# Autodesk Inventor assembly: ant-backlash
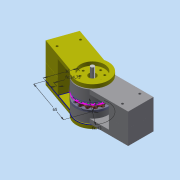
[picture p0: Inventor's stored thumbnail of the model, 180x180]
Saved by Autodesk Inventor 2020.2 (Build 242310000, 310)
## iProperties
Created: 2018-11-17
Part Number: ant-backlash
Document SubType Name: Assembly
Designer: paulg
Author: paulg
## Documents named in this file (13)
- D:\Projects\MiniBot\CAD\cycloidal gear\source\ant-backlash.iam
- D:\Projects\MiniBot\CAD\cycloidal gear\source\ab_output_in.ipt
- D:\Projects\MiniBot\CAD\cycloidal gear\source\ab_output_out.ipt
- D:\Projects\MiniBot\CAD\cycloidal gear\source\Main_equation_fixed_9mm.ipt
- D:\Projects\MiniBot\CAD\cycloidal gear\source\offset 6id 12- od 9mm.ipt
- D:\Projects\MiniBot\CAD\cycloidal gear\source\45x58x7 bearing.ipt
- D:\Projects\MiniBot\CAD\cycloidal gear\source\encoder in 6809_ab.ipt
- D:\Projects\MiniBot\CAD\cycloidal gear\source\motor_6809_ab.ipt
- D:\Projects\MiniBot\CAD\cycloidal gear\source\motor_shaft-ab.ipt
- D:\Projects\MiniBot\CAD\cycloidal gear\source\12x6x4 bearing.ipt
- D:\Projects\MiniBot\CAD\cycloidal gear\source\18x12x4 bearing.ipt
- D:\Projects\MiniBot\CAD\cycloidal gear\source\8x5x2.5 bearing.ipt
- D:\Projects\MiniBot\CAD\cycloidal gear\source\inner_rods.ipt
## Components (40 placed, 12 different names)
1. ab_output_in:1 — Insert:1, Insert:2, Passend:16, Passend:17
2. ab_output_out:1 — Insert:1, Insert:11, Flush:2, Passend:16, Passend:17, Passend:18
3. ab_output_out:2 — Insert:2, Insert:8, Flush:2, Passend:18
4. Main_equation_fixed_9mm:1 — Insert:17, Insert:25, Passend:10, Passend:12
5. offset 6id 12- od 9mm:1 — Insert:5, Insert:22, Insert:24, Passend:6, Passend:7, Passend:8, Passend:9, Passend:10, Passend:11, Passend:12, Passend:13, Passend:14
6. Main_equation_fixed_9mm:2 — Insert:5, Insert:16, Insert:19, Insert:21, Passend:11, Passend:15
7. encoder in 6809_ab:1 — Insert:6, Passend:19
8. motor_6809_ab:1 — Insert:12, Einfügen:23, Passend:5, Passend:19
9. 45x58x7 bearing:1 — Insert:11, Insert:12
10. 45x58x7 bearing:2 — Insert:6, Insert:8
11. motor_shaft-ab:1 — Passend:3, Passend:5, Passend:6
12. 12x6x4 bearing:1 — Passend:3, Passend:7
13. 18x12x4 bearing:1 — Insert:19, Passend:8, Passend:14
14. 18x12x4 bearing:2 — Insert:21, Passend:9, Passend:13, Passend:15
15. 18x12x4 bearing:3 — Insert:22
16. 18x12x4 bearing:4 — Insert:24, Insert:25
17. 8x5x2.5 bearing:2 — Insert:16
18. 8x5x2.5 bearing:3
19. 8x5x2.5 bearing:4
20. 8x5x2.5 bearing:5
21. 8x5x2.5 bearing:6
22. 8x5x2.5 bearing:7
23. 8x5x2.5 bearing:8
24. 8x5x2.5 bearing:9
25. 8x5x2.5 bearing:1 — Insert:17
26. 8x5x2.5 bearing:10
27. 8x5x2.5 bearing:11
28. 8x5x2.5 bearing:12
29. 8x5x2.5 bearing:13
30. 8x5x2.5 bearing:14
31. 8x5x2.5 bearing:15
32. 8x5x2.5 bearing:16
33. inner_rods:1 — Einfügen:23
34. inner_rods:2
35. inner_rods:3
36. inner_rods:4
37. inner_rods:5
38. inner_rods:6
39. inner_rods:7
40. inner_rods:8
## Component patterns: (8 elements, first: 8x5x2.5 bearing:2), (8 elements, first: 8x5x2.5 bearing:1), (8 elements, first: inner_rods:1)
## Relationships (32: Mate 16, Insert 15, Flush 1)
- Insert:1: ab_output_in:1 ↔ ab_output_out:1
- Insert:2: ab_output_in:1 ↔ ab_output_out:2
- Insert:5 (0.5 mm): offset 6id 12- od 9mm:1 ↔ Main_equation_fixed_9mm:2
- Insert:6: encoder in 6809_ab:1 ↔ 45x58x7 bearing:2
- Insert:8: ab_output_out:2 ↔ 45x58x7 bearing:2
- Insert:11: ab_output_out:1 ↔ 45x58x7 bearing:1
- Insert:12: motor_6809_ab:1 ↔ 45x58x7 bearing:1
- Insert:16 (1 mm): Main_equation_fixed_9mm:2 ↔ 8x5x2.5 bearing:2
- Insert:17 (1 mm): Main_equation_fixed_9mm:1 ↔ 8x5x2.5 bearing:1
- Insert:19: Main_equation_fixed_9mm:2 ↔ 18x12x4 bearing:1
- Insert:21: Main_equation_fixed_9mm:2 ↔ 18x12x4 bearing:2
- Insert:22: offset 6id 12- od 9mm:1 ↔ 18x12x4 bearing:3
- Einfügen:23 [Insert] (-5 mm): motor_6809_ab:1 ↔ inner_rods:1
- Insert:24: offset 6id 12- od 9mm:1 ↔ 18x12x4 bearing:4
- Insert:25: Main_equation_fixed_9mm:1 ↔ 18x12x4 bearing:4
- Flush:2: ab_output_out:1 ↔ ab_output_out:2
- Passend:3 [Mate]: motor_shaft-ab:1 ↔ 12x6x4 bearing:1
- Passend:5 [Mate]: motor_6809_ab:1 ↔ motor_shaft-ab:1
- Passend:6 [Mate]: offset 6id 12- od 9mm:1 ↔ motor_shaft-ab:1
- Passend:7 [Mate]: offset 6id 12- od 9mm:1 ↔ 12x6x4 bearing:1
- Passend:8 [Mate]: offset 6id 12- od 9mm:1 ↔ 18x12x4 bearing:1
- Passend:9 [Mate]: offset 6id 12- od 9mm:1 ↔ 18x12x4 bearing:2
- Passend:10 [Mate]: Main_equation_fixed_9mm:1 ↔ offset 6id 12- od 9mm:1
- Passend:11 [Mate]: offset 6id 12- od 9mm:1 ↔ Main_equation_fixed_9mm:2
- Passend:12 [Mate]: Main_equation_fixed_9mm:1 ↔ offset 6id 12- od 9mm:1
- Passend:13 [Mate]: offset 6id 12- od 9mm:1 ↔ 18x12x4 bearing:2
- Passend:14 [Mate]: offset 6id 12- od 9mm:1 ↔ 18x12x4 bearing:1
- Passend:15 [Mate]: Main_equation_fixed_9mm:2 ↔ 18x12x4 bearing:2
- Passend:16 [Mate]: ab_output_in:1 ↔ ab_output_out:1
- Passend:17 [Mate]: ab_output_in:1 ↔ ab_output_out:1
- Passend:18 [Mate]: ab_output_out:1 ↔ ab_output_out:2
- Passend:19 [Mate]: encoder in 6809_ab:1 ↔ motor_6809_ab:1
